# Autodesk Inventor assembly: Gehäuse
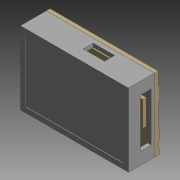
[picture p0: Inventor's stored thumbnail of the model, 180x180]
Saved by Autodesk Inventor 2014 (Build 180170000, 170)
## iProperties
Created: 2016-07-08
Part Number: Gehäuse
Document SubType Name: Assembly
Designer: cem
Author: cem
## Documents named in this file (4)
- C:\development\AnySense\Hardware\Gehäuse\Gehäuse.iam
- C:\development\AnySense\Hardware\Gehäuse\Platine.ipt
- C:\development\AnySense\Hardware\Gehäuse\Boden.ipt
- C:\development\AnySense\Hardware\Gehäuse\Deckel.ipt
## Components (3 placed, 3 different names)
1. Platine:1 — Fluchtend:3, Fluchtend:4, Fluchtend:5, Passend:1, Fluchtend:15
2. Boden:1 — Fluchtend:3, Fluchtend:4, Fluchtend:5, Passend:1, Fluchtend:6, Fluchtend:7, Fluchtend:8, Fluchtend:10, Fluchtend:11, Fluchtend:12, Fluchtend:13
3. Deckel:1 — Fluchtend:6, Fluchtend:7, Fluchtend:8, Fluchtend:10, Fluchtend:11, Fluchtend:12, Fluchtend:13, Fluchtend:15
## Relationships (12: Flush 11, Mate 1)
- Fluchtend:3 [Flush]: Platine:1 ↔ Boden:1
- Fluchtend:4 [Flush] (2 mm): Platine:1 ↔ Boden:1
- Fluchtend:5 [Flush] (1.5 mm): Platine:1 ↔ Boden:1
- Passend:1 [Mate]: Platine:1 ↔ Boden:1
- Fluchtend:6 [Flush]: Boden:1 ↔ Deckel:1
- Fluchtend:7 [Flush]: Boden:1 ↔ Deckel:1
- Fluchtend:8 [Flush]: Boden:1 ↔ Deckel:1
- Fluchtend:10 [Flush]: Boden:1 ↔ Deckel:1
- Fluchtend:11 [Flush]: Boden:1 ↔ Deckel:1
- Fluchtend:12 [Flush]: Boden:1 ↔ Deckel:1
- Fluchtend:13 [Flush]: Boden:1 ↔ Deckel:1
- Fluchtend:15 [Flush] (-0.3 mm): Platine:1 ↔ Deckel:1
